# Autodesk Inventor assembly: SPE0V1 Ensamble General
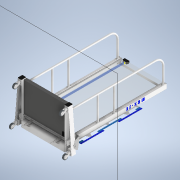
[picture p0: Inventor's stored thumbnail of the model, 180x180]
Saved by Autodesk Inventor 2021.2 (Build 252289000, 289)
## iProperties
Created: 2026-05-12
Part Number: SPE0V1 Ensamble General
Document SubType Name: Assembly
Designer: nelso
Author: nelso
## Documents named in this file (17)
- C:\Users\nelso\Documents\Escritorio\Soporte-Paciente-Espinografia\Workspace\SPE0V1 Ensamble General.iam
- C:\Users\nelso\Documents\Escritorio\Soporte-Paciente-Espinografia\Workspace\SPE1V1 Estructura.iam
- C:\Users\nelso\Documents\Escritorio\Soporte-Paciente-Espinografia\Workspace\SPE2V1 Baranda.iam
- C:\Users\nelso\Documents\Escritorio\Soporte-Paciente-Espinografia\Workspace\DIN933M8X1.25L20C.ipt
- C:\Users\nelso\Documents\Escritorio\Soporte-Paciente-Espinografia\Workspace\DIN125-A8,4C.ipt
- C:\Users\nelso\Documents\Escritorio\Soporte-Paciente-Espinografia\Workspace\Logo.ipt
- C:\Users\nelso\Documents\Escritorio\Soporte-Paciente-Espinografia\Workspace\SPE31V1 Bisagra.iam
- C:\Users\nelso\Documents\Escritorio\Soporte-Paciente-Espinografia\Workspace\DIN 555A5C.ipt
- C:\Users\nelso\Documents\Escritorio\Soporte-Paciente-Espinografia\Workspace\DIN125-A6C.ipt
- C:\Users\nelso\Documents\Escritorio\Soporte-Paciente-Espinografia\Workspace\DIN912-M6X1L16P.ipt
- C:\Users\nelso\Documents\Escritorio\Soporte-Paciente-Espinografia\Workspace\SPE42 Base Paciente.iam
- C:\Users\nelso\Documents\Escritorio\Soporte-Paciente-Espinografia\Workspace\SPE44V1 Acrilico Paciente.iam
- C:\Users\nelso\Documents\Escritorio\Soporte-Paciente-Espinografia\Workspace\RFPLUS8PO300.ipt
- C:\Users\nelso\Documents\Escritorio\Soporte-Paciente-Espinografia\Workspace\SPE48V2 Roldana Acrilico.iam
- C:\Users\nelso\Documents\Escritorio\Soporte-Paciente-Espinografia\Workspace\SP56V1 Chapa Detectores.ipt
- C:\Users\nelso\Documents\Escritorio\Soporte-Paciente-Espinografia\Workspace\PinturaDetectores.ipt
- C:\Users\nelso\Documents\Escritorio\Soporte-Paciente-Espinografia\Workspace\SP57V1 Felpa Detectores.ipt
## Components (85 placed, 16 different names)
1. SPE1V1 Estructura:1 [sub-assembly] — Coincidencia:100, Coincidencia:117, Nivelación:14, Nivelación:15, Mate:236, Mate:237, Mate:331, Mate:332, Mate:333, Mate:337, Mate:338, Mate:339, Mate:340, Mate:341, Mate:342, Mate:513, Mate:514, Mate:516, Mate:517, Mate:524, Mate:526, Flush:62, Flush:63, Flush:64, Mate:528, Mate:529, Mate:530, Mate:531, Mate:532, Mate:533, Flush:65, Flush:66, Flush:67, Flush:68, Angle:1, Flush:69, Mate:540, Mate:541, Mate:547, Mate:550
2. SPE2V1 Baranda:2 [sub-assembly] — Coincidencia:100, Coincidencia:109, Coincidencia:110, Coincidencia:111, Coincidencia:112, Mate:134, Mate:135, Mate:136, Mate:137, Mate:138, Mate:139, Mate:140, Mate:141, Mate:142, Mate:143, Mate:144, Mate:145, Mate:168, Mate:169, Mate:170, Mate:171, Mate:172, Mate:173, Mate:533
3. SPE2V1 Baranda:3 [sub-assembly] — Mate:118, Mate:119, Mate:120, Mate:121, Mate:122, Mate:123, Mate:124, Mate:125, Mate:126, Mate:127, Mate:128, Mate:129, Mate:130, Mate:131, Mate:132, Mate:133, Mate:147, Mate:149, Mate:156, Mate:157, Mate:158, Mate:159, Mate:160, Mate:236, Mate:530
4. DIN933M8X1.25L20C:1 — Coincidencia:113, Coincidencia:114, Mate:532
5. DIN125-A8,4C:1 — Coincidencia:109, Coincidencia:110, Coincidencia:115, Coincidencia:116
6. DIN125-A8,4C:2 — Coincidencia:111, Coincidencia:112, Coincidencia:113, Coincidencia:114
7. DIN933M8X1.25L20C:2 — Coincidencia:115, Coincidencia:116, Mate:531
8. Logo:1 — Coincidencia:117, Nivelación:14, Nivelación:15
9. DIN125-A8,4C:3 — Mate:144, Mate:145, Mate:162
10. DIN125-A8,4C:4 — Mate:142, Mate:143, Mate:163
11. DIN125-A8,4C:5 — Mate:140, Mate:141, Mate:164
12. DIN125-A8,4C:6 — Mate:138, Mate:139, Mate:165
13. DIN125-A8,4C:7 — Mate:135, Mate:136, Mate:167
14. DIN125-A8,4C:8 — Mate:134, Mate:137, Mate:166
15. DIN125-A8,4C:9 — Mate:130, Mate:132, Mate:155
16. DIN125-A8,4C:10 — Mate:131, Mate:133, Mate:154
17. DIN125-A8,4C:11 — Mate:128, Mate:129, Mate:153
18. DIN125-A8,4C:12 — Mate:126, Mate:127, Mate:152
19. DIN125-A8,4C:13 — Mate:122, Mate:123, Mate:150
20. DIN125-A8,4C:14 — Mate:124, Mate:125, Mate:151
21. DIN125-A8,4C:15 — Mate:120, Mate:121, Mate:148
22. DIN125-A8,4C:16 — Mate:118, Mate:119, Mate:146
23. DIN933M8X1.25L20C:3 — Mate:162, Mate:168
24. DIN933M8X1.25L20C:4 — Mate:163, Mate:169
25. DIN933M8X1.25L20C:5 — Mate:164, Mate:170
26. DIN933M8X1.25L20C:6 — Mate:165, Mate:171
27. DIN933M8X1.25L20C:7 — Mate:166, Mate:172, Mate:534
28. DIN933M8X1.25L20C:8 — Mate:167, Mate:173, Mate:535
29. DIN933M8X1.25L20C:9 — Mate:155, Mate:156, Mate:537
30. DIN933M8X1.25L20C:10 — Mate:154, Mate:157, Mate:536
31. DIN933M8X1.25L20C:11 — Mate:153, Mate:159
32. DIN933M8X1.25L20C:12 — Mate:152, Mate:158
33. DIN933M8X1.25L20C:13 — Mate:151, Mate:160
34. DIN933M8X1.25L20C:14 — Mate:150, Mate:237
35. DIN933M8X1.25L20C:15 — Mate:148, Mate:149, Mate:529
36. DIN933M8X1.25L20C:16 — Mate:146, Mate:147, Mate:528
37. SPE31V1 Bisagra:1 [sub-assembly] — Mate:333, Mate:341, Mate:342, Mate:468, Mate:469, Mate:470, Mate:471, Mate:472, Mate:473, Mate:474, Mate:475
38. SPE31V1 Bisagra:2 [sub-assembly] — Mate:331, Mate:337, Mate:338, Mate:452, Mate:453, Mate:454, Mate:455, Mate:456, Mate:457, Mate:458, Mate:459
39. SPE31V1 Bisagra:3 [sub-assembly] — Mate:332, Mate:339, Mate:340, Mate:460, Mate:461, Mate:462, Mate:463, Mate:464, Mate:465, Mate:466, Mate:467
40. DIN912-M6X1L16P:2 — Mate:452, Mate:454, Mate:522
41. DIN912-M6X1L16P:3 — Mate:453, Mate:455, Mate:523, Mate:525
42. DIN912-M6X1L16P:4 — Mate:456, Mate:457, Mate:506
43. DIN912-M6X1L16P:5 — Mate:458, Mate:459, Mate:507
44. DIN912-M6X1L16P:6 — Mate:460, Mate:464, Mate:518
45. DIN912-M6X1L16P:7 — Mate:462, Mate:466, Mate:508
46. DIN912-M6X1L16P:8 — Mate:461, Mate:465, Mate:519
47. DIN912-M6X1L16P:9 — Mate:463, Mate:467, Mate:509
48. DIN912-M6X1L16P:10 — Mate:469, Mate:473, Mate:521
49. DIN912-M6X1L16P:11 — Mate:468, Mate:472, Mate:520
50. DIN912-M6X1L16P:12 — Mate:470, Mate:474, Mate:510
51. DIN912-M6X1L16P:13 — Mate:471, Mate:475, Mate:511
52. DIN 555A5C:1 — Mate:476, Mate:488, Mate:519
53. DIN 555A5C:2 — Mate:477, Mate:489, Mate:506
54. DIN 555A5C:3 — Mate:478, Mate:523
55. DIN 555A5C:4 — Mate:479, Mate:491, Mate:509
56. DIN 555A5C:5 — Mate:480, Mate:492, Mate:518
57. DIN 555A5C:6 — Mate:481, Mate:493, Mate:508
58. DIN 555A5C:7 — Mate:482, Mate:494, Mate:521
59. DIN 555A5C:8 — Mate:483, Mate:495, Mate:510
60. DIN 555A5C:9 — Mate:485, Mate:497, Mate:522
61. DIN 555A5C:10 — Mate:484, Mate:496, Mate:507
62. DIN 555A5C:11 — Mate:486, Mate:498, Mate:511
63. DIN 555A5C:12 — Mate:487, Mate:499, Mate:520
64. DIN125-A6C:1 — Mate:476, Mate:488, Mate:513
65. DIN125-A6C:2 — Mate:477, Mate:489
66. DIN125-A6C:3 — Mate:478, Mate:524, Mate:525
67. DIN125-A6C:4 — Mate:479, Mate:491
68. DIN125-A6C:5 — Mate:480, Mate:492, Mate:514
69. DIN125-A6C:6 — Mate:481, Mate:493
70. DIN125-A6C:7 — Mate:482, Mate:494, Mate:517
71. DIN125-A6C:8 — Mate:483, Mate:495
72. DIN125-A6C:9 — Mate:484, Mate:496
73. DIN125-A6C:10 — Mate:485, Mate:497, Mate:526
74. DIN125-A6C:11 — Mate:486, Mate:498
75. DIN125-A6C:12 — Mate:487, Mate:499, Mate:516
76. SPE42 Base Paciente:1 [sub-assembly] — Angle:1
77. SPE44V1 Acrilico Paciente:1 [sub-assembly] — Mate:540, Mate:541, Mate:542, Flush:70, Mate:543
78. RFPLUS8PO300:1 — Mate:534, Flush:67
79. RFPLUS8PO300:2 — Mate:535, Flush:68
80. RFPLUS8PO300:3 — Mate:536, Flush:65
81. RFPLUS8PO300:4 — Mate:537, Flush:66
82. SPE48V2 Roldana Acrilico:1 [sub-assembly] — Mate:542, Flush:70, Mate:543
83. SP56V1 Chapa Detectores:1 — Mate:546, Flush:71, Flush:72, Mate:547, Mate:548, Flush:73, Mate:549
84. PinturaDetectores:1 — Mate:546, Flush:71, Flush:72
85. SP57V1 Felpa Detectores:1 — Mate:548, Flush:73, Mate:549, Mate:550
## Relationships (190: Mate 173, Flush 16, Angle 1)
- Coincidencia:100 [Mate]: SPE1V1 Estructura:1 ↔ SPE2V1 Baranda:2
- Coincidencia:109 [Mate]: SPE2V1 Baranda:2 ↔ DIN125-A8,4C:1
- Coincidencia:110 [Mate]: SPE2V1 Baranda:2 ↔ DIN125-A8,4C:1
- Coincidencia:111 [Mate]: SPE2V1 Baranda:2 ↔ DIN125-A8,4C:2
- Coincidencia:112 [Mate]: SPE2V1 Baranda:2 ↔ DIN125-A8,4C:2
- Coincidencia:113 [Mate]: DIN933M8X1.25L20C:1 ↔ DIN125-A8,4C:2
- Coincidencia:114 [Mate]: DIN933M8X1.25L20C:1 ↔ DIN125-A8,4C:2
- Coincidencia:115 [Mate]: DIN125-A8,4C:1 ↔ DIN933M8X1.25L20C:2
- Coincidencia:116 [Mate]: DIN125-A8,4C:1 ↔ DIN933M8X1.25L20C:2
- Coincidencia:117 [Mate]: SPE1V1 Estructura:1 ↔ Logo:1
- Nivelación:14 [Flush] (8 mm): SPE1V1 Estructura:1 ↔ Logo:1
- Nivelación:15 [Flush] (400 mm): SPE1V1 Estructura:1 ↔ Logo:1
- Mate:118: SPE2V1 Baranda:3 ↔ DIN125-A8,4C:16
- Mate:119: SPE2V1 Baranda:3 ↔ DIN125-A8,4C:16
- Mate:120: SPE2V1 Baranda:3 ↔ DIN125-A8,4C:15
- Mate:121: SPE2V1 Baranda:3 ↔ DIN125-A8,4C:15
- Mate:122: SPE2V1 Baranda:3 ↔ DIN125-A8,4C:13
- Mate:123: SPE2V1 Baranda:3 ↔ DIN125-A8,4C:13
- Mate:124: SPE2V1 Baranda:3 ↔ DIN125-A8,4C:14
- Mate:125: SPE2V1 Baranda:3 ↔ DIN125-A8,4C:14
- Mate:126: SPE2V1 Baranda:3 ↔ DIN125-A8,4C:12
- Mate:127: SPE2V1 Baranda:3 ↔ DIN125-A8,4C:12
- Mate:128: SPE2V1 Baranda:3 ↔ DIN125-A8,4C:11
- Mate:129: SPE2V1 Baranda:3 ↔ DIN125-A8,4C:11
- Mate:130: SPE2V1 Baranda:3 ↔ DIN125-A8,4C:9
- Mate:131: SPE2V1 Baranda:3 ↔ DIN125-A8,4C:10
- Mate:132: SPE2V1 Baranda:3 ↔ DIN125-A8,4C:9
- Mate:133: SPE2V1 Baranda:3 ↔ DIN125-A8,4C:10
- Mate:134: SPE2V1 Baranda:2 ↔ DIN125-A8,4C:8
- Mate:135: SPE2V1 Baranda:2 ↔ DIN125-A8,4C:7
- Mate:136: SPE2V1 Baranda:2 ↔ DIN125-A8,4C:7
- Mate:137: SPE2V1 Baranda:2 ↔ DIN125-A8,4C:8
- Mate:138: SPE2V1 Baranda:2 ↔ DIN125-A8,4C:6
- Mate:139: SPE2V1 Baranda:2 ↔ DIN125-A8,4C:6
- Mate:140: SPE2V1 Baranda:2 ↔ DIN125-A8,4C:5
- Mate:141: SPE2V1 Baranda:2 ↔ DIN125-A8,4C:5
- Mate:142: SPE2V1 Baranda:2 ↔ DIN125-A8,4C:4
- Mate:143: SPE2V1 Baranda:2 ↔ DIN125-A8,4C:4
- Mate:144: SPE2V1 Baranda:2 ↔ DIN125-A8,4C:3
- Mate:145: SPE2V1 Baranda:2 ↔ DIN125-A8,4C:3
- Mate:146: DIN125-A8,4C:16 ↔ DIN933M8X1.25L20C:16
- Mate:147: SPE2V1 Baranda:3 ↔ DIN933M8X1.25L20C:16
- Mate:148: DIN125-A8,4C:15 ↔ DIN933M8X1.25L20C:15
- Mate:149: SPE2V1 Baranda:3 ↔ DIN933M8X1.25L20C:15
- Mate:150: DIN125-A8,4C:13 ↔ DIN933M8X1.25L20C:14
- Mate:151: DIN125-A8,4C:14 ↔ DIN933M8X1.25L20C:13
- Mate:152: DIN125-A8,4C:12 ↔ DIN933M8X1.25L20C:12
- Mate:153: DIN125-A8,4C:11 ↔ DIN933M8X1.25L20C:11
- Mate:154: DIN125-A8,4C:10 ↔ DIN933M8X1.25L20C:10
- Mate:155: DIN125-A8,4C:9 ↔ DIN933M8X1.25L20C:9
- Mate:156: SPE2V1 Baranda:3 ↔ DIN933M8X1.25L20C:9
- Mate:157: SPE2V1 Baranda:3 ↔ DIN933M8X1.25L20C:10
- Mate:158: SPE2V1 Baranda:3 ↔ DIN933M8X1.25L20C:12
- Mate:159: SPE2V1 Baranda:3 ↔ DIN933M8X1.25L20C:11
- Mate:160: SPE2V1 Baranda:3 ↔ DIN933M8X1.25L20C:13
- Mate:162: DIN125-A8,4C:3 ↔ DIN933M8X1.25L20C:3
- Mate:163: DIN125-A8,4C:4 ↔ DIN933M8X1.25L20C:4
- Mate:164: DIN125-A8,4C:5 ↔ DIN933M8X1.25L20C:5
- Mate:165: DIN125-A8,4C:6 ↔ DIN933M8X1.25L20C:6
- Mate:166: DIN125-A8,4C:8 ↔ DIN933M8X1.25L20C:7
- Mate:167: DIN125-A8,4C:7 ↔ DIN933M8X1.25L20C:8
- Mate:168: SPE2V1 Baranda:2 ↔ DIN933M8X1.25L20C:3
- Mate:169: SPE2V1 Baranda:2 ↔ DIN933M8X1.25L20C:4
- Mate:170: SPE2V1 Baranda:2 ↔ DIN933M8X1.25L20C:5
- Mate:171: SPE2V1 Baranda:2 ↔ DIN933M8X1.25L20C:6
- Mate:172: SPE2V1 Baranda:2 ↔ DIN933M8X1.25L20C:7
- Mate:173: SPE2V1 Baranda:2 ↔ DIN933M8X1.25L20C:8
- Mate:236: SPE1V1 Estructura:1 ↔ SPE2V1 Baranda:3
- Mate:237: SPE1V1 Estructura:1 ↔ DIN933M8X1.25L20C:14
- [Mate]: SPE1V1 Estructura:1 ↔ SPE44V1 Acrilico Paciente:1
- [Flush]: SPE1V1 Estructura:1 ↔ SPE44V1 Acrilico Paciente:1
- Mate:331: SPE1V1 Estructura:1 ↔ SPE31V1 Bisagra:2
- Mate:332: SPE1V1 Estructura:1 ↔ SPE31V1 Bisagra:3
- Mate:333: SPE1V1 Estructura:1 ↔ SPE31V1 Bisagra:1
- Mate:337: SPE1V1 Estructura:1 ↔ SPE31V1 Bisagra:2
- Mate:338: SPE1V1 Estructura:1 ↔ SPE31V1 Bisagra:2
- Mate:339: SPE1V1 Estructura:1 ↔ SPE31V1 Bisagra:3
- Mate:340: SPE1V1 Estructura:1 ↔ SPE31V1 Bisagra:3
- Mate:341: SPE1V1 Estructura:1 ↔ SPE31V1 Bisagra:1
- Mate:342: SPE1V1 Estructura:1 ↔ SPE31V1 Bisagra:1
- [Mate]: SPE31V1 Bisagra:3 ↔ SPE42 Base Paciente:1
- [Mate]: SPE31V1 Bisagra:2 ↔ SPE42 Base Paciente:1
- [Mate]: SPE31V1 Bisagra:1 ↔ SPE42 Base Paciente:1
- [Mate]: SPE31V1 Bisagra:2 ↔ SPE42 Base Paciente:1
- [Mate]: SPE31V1 Bisagra:1 ↔ SPE42 Base Paciente:1
- Mate:452: SPE31V1 Bisagra:2 ↔ DIN912-M6X1L16P:2
- Mate:453: SPE31V1 Bisagra:2 ↔ DIN912-M6X1L16P:3
- Mate:454: SPE31V1 Bisagra:2 ↔ DIN912-M6X1L16P:2
- Mate:455: SPE31V1 Bisagra:2 ↔ DIN912-M6X1L16P:3
- Mate:456: SPE31V1 Bisagra:2 ↔ DIN912-M6X1L16P:4
- Mate:457: SPE31V1 Bisagra:2 ↔ DIN912-M6X1L16P:4
- Mate:458: SPE31V1 Bisagra:2 ↔ DIN912-M6X1L16P:5
- Mate:459: SPE31V1 Bisagra:2 ↔ DIN912-M6X1L16P:5
- Mate:460: SPE31V1 Bisagra:3 ↔ DIN912-M6X1L16P:6
- Mate:461: SPE31V1 Bisagra:3 ↔ DIN912-M6X1L16P:8
- Mate:462: SPE31V1 Bisagra:3 ↔ DIN912-M6X1L16P:7
- Mate:463: SPE31V1 Bisagra:3 ↔ DIN912-M6X1L16P:9
- Mate:464: SPE31V1 Bisagra:3 ↔ DIN912-M6X1L16P:6
- Mate:465: SPE31V1 Bisagra:3 ↔ DIN912-M6X1L16P:8
- Mate:466: SPE31V1 Bisagra:3 ↔ DIN912-M6X1L16P:7
- Mate:467: SPE31V1 Bisagra:3 ↔ DIN912-M6X1L16P:9
- Mate:468: SPE31V1 Bisagra:1 ↔ DIN912-M6X1L16P:11
- Mate:469: SPE31V1 Bisagra:1 ↔ DIN912-M6X1L16P:10
- Mate:470: SPE31V1 Bisagra:1 ↔ DIN912-M6X1L16P:12
- Mate:471: SPE31V1 Bisagra:1 ↔ DIN912-M6X1L16P:13
- Mate:472: SPE31V1 Bisagra:1 ↔ DIN912-M6X1L16P:11
- Mate:473: SPE31V1 Bisagra:1 ↔ DIN912-M6X1L16P:10
- Mate:474: SPE31V1 Bisagra:1 ↔ DIN912-M6X1L16P:12
- Mate:475: SPE31V1 Bisagra:1 ↔ DIN912-M6X1L16P:13
- Mate:476: DIN 555A5C:1 ↔ DIN125-A6C:1
- Mate:477: DIN 555A5C:2 ↔ DIN125-A6C:2
- Mate:478: DIN 555A5C:3 ↔ DIN125-A6C:3
- Mate:479: DIN 555A5C:4 ↔ DIN125-A6C:4
- Mate:480: DIN 555A5C:5 ↔ DIN125-A6C:5
- Mate:481: DIN 555A5C:6 ↔ DIN125-A6C:6
- Mate:482: DIN 555A5C:7 ↔ DIN125-A6C:7
- Mate:483: DIN 555A5C:8 ↔ DIN125-A6C:8
- Mate:484: DIN 555A5C:10 ↔ DIN125-A6C:9
- Mate:485: DIN 555A5C:9 ↔ DIN125-A6C:10
- Mate:486: DIN 555A5C:11 ↔ DIN125-A6C:11
- Mate:487: DIN 555A5C:12 ↔ DIN125-A6C:12
- Mate:488: DIN 555A5C:1 ↔ DIN125-A6C:1
- Mate:489: DIN 555A5C:2 ↔ DIN125-A6C:2
- Mate:491: DIN 555A5C:4 ↔ DIN125-A6C:4
- Mate:492: DIN 555A5C:5 ↔ DIN125-A6C:5
- Mate:493: DIN 555A5C:6 ↔ DIN125-A6C:6
- Mate:494: DIN 555A5C:7 ↔ DIN125-A6C:7
- Mate:495: DIN 555A5C:8 ↔ DIN125-A6C:8
- Mate:496: DIN 555A5C:10 ↔ DIN125-A6C:9
- Mate:497: DIN 555A5C:9 ↔ DIN125-A6C:10
- Mate:498: DIN 555A5C:11 ↔ DIN125-A6C:11
- Mate:499: DIN 555A5C:12 ↔ DIN125-A6C:12
- [Mate]: DIN125-A6C:2 ↔ SPE42 Base Paciente:1
- [Mate]: DIN125-A6C:9 ↔ SPE42 Base Paciente:1
- [Mate]: DIN125-A6C:4 ↔ SPE42 Base Paciente:1
- [Mate]: DIN125-A6C:6 ↔ SPE42 Base Paciente:1
- [Mate]: DIN125-A6C:8 ↔ SPE42 Base Paciente:1
- [Mate]: DIN125-A6C:11 ↔ SPE42 Base Paciente:1
- Mate:506: DIN912-M6X1L16P:4 ↔ DIN 555A5C:2
- Mate:507: DIN912-M6X1L16P:5 ↔ DIN 555A5C:10
- Mate:508: DIN912-M6X1L16P:7 ↔ DIN 555A5C:6
- Mate:509: DIN912-M6X1L16P:9 ↔ DIN 555A5C:4
- Mate:510: DIN912-M6X1L16P:12 ↔ DIN 555A5C:8
- Mate:511: DIN912-M6X1L16P:13 ↔ DIN 555A5C:11
- Mate:513: SPE1V1 Estructura:1 ↔ DIN125-A6C:1
- Mate:514: SPE1V1 Estructura:1 ↔ DIN125-A6C:5
- Mate:516: SPE1V1 Estructura:1 ↔ DIN125-A6C:12
- Mate:517: SPE1V1 Estructura:1 ↔ DIN125-A6C:7
- Mate:518: DIN912-M6X1L16P:6 ↔ DIN 555A5C:5
- Mate:519: DIN912-M6X1L16P:8 ↔ DIN 555A5C:1
- Mate:520: DIN912-M6X1L16P:11 ↔ DIN 555A5C:12
- Mate:521: DIN912-M6X1L16P:10 ↔ DIN 555A5C:7
- Mate:522: DIN912-M6X1L16P:2 ↔ DIN 555A5C:9
- Mate:523: DIN912-M6X1L16P:3 ↔ DIN 555A5C:3
- Mate:524: SPE1V1 Estructura:1 ↔ DIN125-A6C:3
- Mate:525: DIN912-M6X1L16P:3 ↔ DIN125-A6C:3
- Mate:526: SPE1V1 Estructura:1 ↔ DIN125-A6C:10
- [Flush]: SPE1V1 Estructura:1 ↔ SPE44V1 Acrilico Paciente:1
- Flush:62: SPE1V1 Estructura:1
- Flush:63: SPE1V1 Estructura:1
- Flush:64: SPE1V1 Estructura:1
- Mate:528: SPE1V1 Estructura:1 ↔ DIN933M8X1.25L20C:16
- Mate:529: SPE1V1 Estructura:1 ↔ DIN933M8X1.25L20C:15
- Mate:530: SPE1V1 Estructura:1 ↔ SPE2V1 Baranda:3
- Mate:531: SPE1V1 Estructura:1 ↔ DIN933M8X1.25L20C:2
- Mate:532: SPE1V1 Estructura:1 ↔ DIN933M8X1.25L20C:1
- Mate:533: SPE1V1 Estructura:1 ↔ SPE2V1 Baranda:2
- Mate:534: DIN933M8X1.25L20C:7 ↔ RFPLUS8PO300:1
- Mate:535: DIN933M8X1.25L20C:8 ↔ RFPLUS8PO300:2
- Mate:536: DIN933M8X1.25L20C:10 ↔ RFPLUS8PO300:3
- Mate:537: DIN933M8X1.25L20C:9 ↔ RFPLUS8PO300:4
- Flush:65: SPE1V1 Estructura:1 ↔ RFPLUS8PO300:3
- Flush:66: SPE1V1 Estructura:1 ↔ RFPLUS8PO300:4
- Flush:67: SPE1V1 Estructura:1 ↔ RFPLUS8PO300:1
- Flush:68: SPE1V1 Estructura:1 ↔ RFPLUS8PO300:2
- Angle:1 (1 deg): SPE1V1 Estructura:1 ↔ SPE42 Base Paciente:1
- Flush:69 (-211 mm): SPE1V1 Estructura:1
- Mate:540: SPE1V1 Estructura:1 ↔ SPE44V1 Acrilico Paciente:1
- Mate:541: SPE1V1 Estructura:1 ↔ SPE44V1 Acrilico Paciente:1
- Mate:542: SPE44V1 Acrilico Paciente:1 ↔ SPE48V2 Roldana Acrilico:1
- Flush:70: SPE44V1 Acrilico Paciente:1 ↔ SPE48V2 Roldana Acrilico:1
- Mate:543: SPE44V1 Acrilico Paciente:1 ↔ SPE48V2 Roldana Acrilico:1
- Mate:546: SP56V1 Chapa Detectores:1 ↔ PinturaDetectores:1
- Flush:71: SP56V1 Chapa Detectores:1 ↔ PinturaDetectores:1
- Flush:72: SP56V1 Chapa Detectores:1 ↔ PinturaDetectores:1
- Mate:547: SPE1V1 Estructura:1 ↔ SP56V1 Chapa Detectores:1
- Mate:548: SP56V1 Chapa Detectores:1 ↔ SP57V1 Felpa Detectores:1
- Flush:73: SP56V1 Chapa Detectores:1 ↔ SP57V1 Felpa Detectores:1
- Mate:549: SP56V1 Chapa Detectores:1 ↔ SP57V1 Felpa Detectores:1
- Mate:550 (-1 mm): SPE1V1 Estructura:1 ↔ SP57V1 Felpa Detectores:1
